# Autodesk Inventor assembly: Epsilon Grabbers
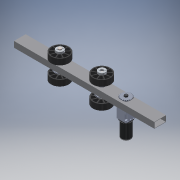
[picture p0: Inventor's stored thumbnail of the model, 180x180]
Saved by Autodesk Inventor 2019 (Build 230136000, 136)
## iProperties
Created: 2019-01-31
Part Number: Epsilon Grabbers
Document SubType Name: Assembly
Designer: josh
Mass: 596.604 g
Surface Area: 3977.42 cm^2
Volume: 596.604 cm^3
Density: 1 g/cm^3
Author: josh
## Documents named in this file (6)
- D:\Synthesis Robots\Epsilon\Epsilon Grabbers\Epsilon Grabbers.iam
- D:\Synthesis Robots\Epsilon\Epsilon Grabbers\Aluminum Channel Arm.ipt
- D:\Synthesis Robots\Epsilon\Epsilon Grabbers\am-0646 S25-22HA-500 Hex Sprocket.ipt
- D:\Synthesis Robots\Epsilon\Epsilon Grabbers\Bag Motor parts\VersaPlanetary_v1_Single_Stage_10_1_with_BAG.iam
- D:\Synthesis Robots\Epsilon\Epsilon Grabbers\Grabbing unit\Eplison gripper 1.iam
- D:\Synthesis Robots\Epsilon\Epsilon Grabbers\Grabbing unit\Epsilon gripper 2.iam
## Components (5 placed, 5 different names)
1. Aluminum Channel Arm:1 — Mate:1, Mate:5, Flush:1, Flush:2, Mate:6, Rotational:1, Rotational:2
2. VersaPlanetary_v1_Single_Stage_10_1_with_BAG:1 [sub-assembly] — Mate:5, Flush:1, Flush:2, Mate:7, Mate:8
3. am-0646 S25-22HA-500 Hex Sprocket:2 — Mate:6, Mate:7, Mate:8
4. Eplison gripper 1:1 [sub-assembly] — Rotational:2
5. Epsilon gripper 2:1 [sub-assembly] — Rotational:1
## Relationships (9: Mate 5, Flush 2, RevoluteJoint 2)
- Mate:1: Aluminum Channel Arm:1
- Mate:5: Aluminum Channel Arm:1 ↔ VersaPlanetary_v1_Single_Stage_10_1_with_BAG:1
- Flush:1 (4.445 mm): Aluminum Channel Arm:1 ↔ VersaPlanetary_v1_Single_Stage_10_1_with_BAG:1
- Flush:2 (127 mm): Aluminum Channel Arm:1 ↔ VersaPlanetary_v1_Single_Stage_10_1_with_BAG:1
- Mate:6: Aluminum Channel Arm:1 ↔ am-0646 S25-22HA-500 Hex Sprocket:2
- Mate:7: VersaPlanetary_v1_Single_Stage_10_1_with_BAG:1 ↔ am-0646 S25-22HA-500 Hex Sprocket:2
- Mate:8: VersaPlanetary_v1_Single_Stage_10_1_with_BAG:1 ↔ am-0646 S25-22HA-500 Hex Sprocket:2
- Rotational:1 [RevoluteJoint]: Aluminum Channel Arm:1 ↔ Epsilon gripper 2:1
- Rotational:2 [RevoluteJoint]: Aluminum Channel Arm:1 ↔ Eplison gripper 1:1
